# Autodesk Inventor assembly: ASY MSC 100.2 Cone tube
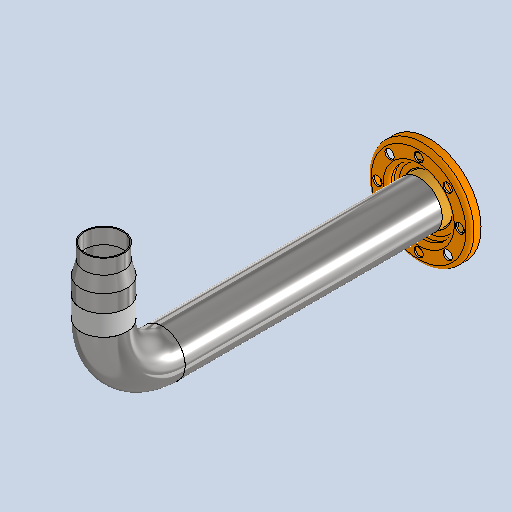
[picture p0: Inventor's stored thumbnail of the model, 512x512]
Saved by Autodesk Inventor 2025 (Build 290162010, 162A)
## iProperties
Created: 2024-08-28
Part Number: ASY MSC 100.2 Cone tube
Document SubType Name: Assembly
Designer: admin
Stock Number: ASY МОО 100.2 конус труба
Author: admin
## Documents named in this file (7)
- C:\Users\pokla\Documents\Inventor\Отстойник осветлитель\Manturovo_Se-clar-Gleb\ASY MSC 100.2 Cone tube.iam
- C:\Users\pokla\Documents\Inventor\Отстойник осветлитель\Manturovo_Se-clar-Gleb\ракета\MSC 104 tube.ipt
- C:\Users\pokla\Documents\Inventor\Отстойник осветлитель\Manturovo_Se-clar-Gleb\ракета\MSC 105 rocket tube 9.ipt
- C:\Users\pokla\Documents\Inventor\Отстойник осветлитель\Manturovo_Se-clar-Gleb\Content Center Files\en-US\JIS B 2312 (1)\JIS B 2312 Concentric Reducer Stainless Steel 80A x 65A x Sch5S.ipt
- C:\Users\pokla\Documents\Inventor\Отстойник осветлитель\Manturovo_Se-clar-Gleb\Content Center Files\en-US\ISO 5251 B 3D\ISO 5251 Bends 3D without straight ends(90 deg) DN80 2 2.ipt
- C:\Users\pokla\Documents\Inventor\Отстойник осветлитель\Manturovo_Se-clar-Gleb\3d party\Stamp flange DIN2642\Stamd flange lapped collar DIN2642\Stamp flange DIN2642-080.ipt
- C:\Users\user\YandexDisk\домашниий пк\Inventor\Manturovo\Manturovo_Se-clar\3d party\Stamp flange DIN2642\Stamd flange lapped collar DIN2642.ipt
## Components (5 placed, 5 different names)
1. МОО 064 ракета труба.ipt:1 — Rigid:2, Rigid:4
2. МОО 069 ракета труба 9.ipt:1 — Rigid:3
3. JIS B 2312 Concentric Reducer Stainless Steel 80A x 65A x Sch5S.ipt:1
4. ISO 5251 Bends 3D without straight ends(90 deg) DN80 2 2.ipt:1 — Rigid:2, Rigid:3
5. Stamp flange DIN2642-080.ipt:1 — Rigid:4
## Relationships (4: WeldJoint 3, RevoluteJoint 1)
- [RevoluteJoint]: МОО 069 ракета труба 9.ipt:1 ↔ JIS B 2312 Concentric Reducer Stainless Steel 80A x 65A x Sch5S.ipt:1
- Rigid:2 [WeldJoint]: МОО 064 ракета труба.ipt:1 ↔ ISO 5251 Bends 3D without straight ends(90 deg) DN80 2 2.ipt:1
- Rigid:3 [WeldJoint]: МОО 069 ракета труба 9.ipt:1 ↔ ISO 5251 Bends 3D without straight ends(90 deg) DN80 2 2.ipt:1
- Rigid:4 [WeldJoint]: МОО 064 ракета труба.ipt:1 ↔ Stamp flange DIN2642-080.ipt:1
